# Autodesk Inventor assembly: Assembly_HoliSheet_v6
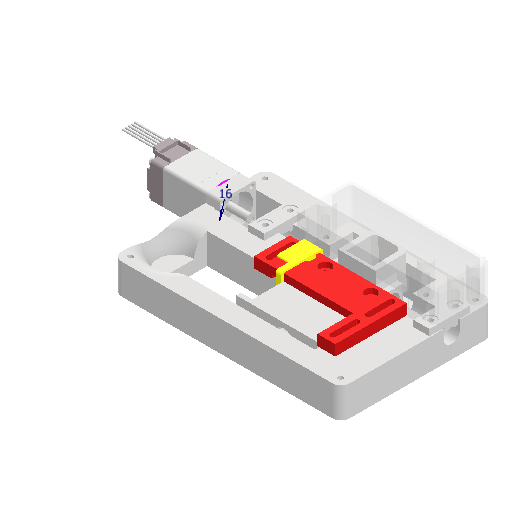
[picture p0: Inventor's stored thumbnail of the model, 512x512]
Saved by Autodesk Inventor 2025.3 (Build 293356000, 356)
## iProperties
Created: 2023-01-07
Part Number: Assembly_HoliSheet_v6
Document SubType Name: Assembly
Designer: diederichbenedict
Author: diederichbenedict
## Documents named in this file (9)
- C:\Users\benir\Documents\HoLiSheet\INVENTOR\Assembly_HoliSheet_v6.iam
- C:\Users\benir\Documents\HoLiSheet\INVENTOR\00_NEMA8.ipt
- C:\Users\benir\Documents\HoLiSheet\INVENTOR\10_Wellplate_base_v6.ipt
- C:\Users\benir\Documents\HoLiSheet\INVENTOR\Holisheet_tubeclamp.ipt
- C:\Users\benir\Documents\HoLiSheet\INVENTOR\HolisheetCageSampleWater.ipt
- C:\Users\benir\Documents\HoLiSheet\INVENTOR\10_Wellplate_base_Lasercover.ipt
- C:\Users\benir\Documents\HoLiSheet\INVENTOR\30_Laser_to_M12Adapter_9,5mm.ipt
- C:\Users\benir\Documents\HoLiSheet\INVENTOR\30_Lightsheet_generator_singlegalvo_1.ipt
- C:\Users\benir\Documents\HoLiSheet\INVENTOR\30_Lightsheet_generator_passive_lid_v1_singlegalvo.ipt
## Components (10 placed, 8 different names)
1. 10_Wellplate_base_v6:1 — Angle:3, Flush:13, Flush:14, Mate:3, Mate:4, Mate:5, Angle:6, Flush:15, Insert:5
2. 00_NEMA8:1 — Angle:3
3. Holisheet_tubeclamp:2
4. HolisheetCageSampleWater:1 — Mate:5, Angle:6
5. Holisheet_tubeclamp:3 — Insert:5
6. 10_Wellplate_base_Lasercover:1 — Flush:13, Flush:14, Insert:6
7. Holisheet_tubeclamp:4 — Insert:6
8. 30_Laser_to_M12Adapter_9,5mm:1 — Insert:4, Angle:5
9. 30_Lightsheet_generator_singlegalvo_1:1 — Insert:3, Angle:4, Mate:3, Insert:4, Angle:5
10. 30_Lightsheet_generator_passive_lid_v1_singlegalvo:1 — Insert:3, Angle:4, Mate:4, Flush:15
## Relationships (14: Angle 4, Insert 4, Flush 3, Mate 3)
- Angle:3 (180 deg): 10_Wellplate_base_v6:1 ↔ 00_NEMA8:1
- Flush:13: 10_Wellplate_base_v6:1 ↔ 10_Wellplate_base_Lasercover:1
- Flush:14: 10_Wellplate_base_v6:1 ↔ 10_Wellplate_base_Lasercover:1
- Insert:3: 30_Lightsheet_generator_singlegalvo_1:1 ↔ 30_Lightsheet_generator_passive_lid_v1_singlegalvo:1
- Angle:4 (180 deg): 30_Lightsheet_generator_singlegalvo_1:1 ↔ 30_Lightsheet_generator_passive_lid_v1_singlegalvo:1
- Mate:3: 10_Wellplate_base_v6:1 ↔ 30_Lightsheet_generator_singlegalvo_1:1
- Mate:4: 10_Wellplate_base_v6:1 ↔ 30_Lightsheet_generator_passive_lid_v1_singlegalvo:1
- Insert:4: 30_Laser_to_M12Adapter_9,5mm:1 ↔ 30_Lightsheet_generator_singlegalvo_1:1
- Angle:5 (270 deg): 30_Laser_to_M12Adapter_9,5mm:1 ↔ 30_Lightsheet_generator_singlegalvo_1:1
- Mate:5: 10_Wellplate_base_v6:1 ↔ HolisheetCageSampleWater:1
- Angle:6 (90 deg): 10_Wellplate_base_v6:1 ↔ HolisheetCageSampleWater:1
- Flush:15 (-5 mm): 10_Wellplate_base_v6:1 ↔ 30_Lightsheet_generator_passive_lid_v1_singlegalvo:1
- Insert:5: 10_Wellplate_base_v6:1 ↔ Holisheet_tubeclamp:3
- Insert:6: 10_Wellplate_base_Lasercover:1 ↔ Holisheet_tubeclamp:4
